# Autodesk Inventor assembly: C6374 170KV Brushless Motor
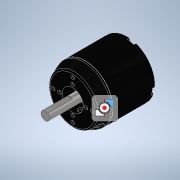
[picture p0: Inventor's stored thumbnail of the model, 180x180]
Saved by Autodesk Inventor 2022 (Build 260153000, 153)
## iProperties
Created: 2022-09-16
Part Number: C6374 170KV Brushless Motor
Document SubType Name: Assembly
Designer: Nathan Cai
Author: Nathan Cai
## Documents named in this file (4)
- C:\Users\Nathan Cai\Documents\Inventor\Asorted Parts\C6374 170KV Brushless Motor\C6374 170KV Brushless Motor.iam
- C:\Users\Nathan Cai\Documents\Inventor\Asorted Parts\C6374 170KV Brushless Motor\Shaft.ipt
- C:\Users\Nathan Cai\Documents\Inventor\Asorted Parts\C6374 170KV Brushless Motor\Base.ipt
- C:\Users\Nathan Cai\Documents\Inventor\Asorted Parts\C6374 170KV Brushless Motor\Can.ipt
## Components (3 placed, 3 different names)
1. Shaft:1 — Flush:1, Mate:2
2. Base:1 — Mate:1, Flush:1, Mate:2, Mate:3
3. Can:1 — Mate:1, Mate:3
## Relationships (4: Mate 3, Flush 1)
- Mate:1: Base:1 ↔ Can:1
- Flush:1 (-31 mm): Shaft:1 ↔ Base:1
- Mate:2: Shaft:1 ↔ Base:1
- Mate:3 (0.25 mm): Base:1 ↔ Can:1
